# Autodesk Inventor assembly: for_bool
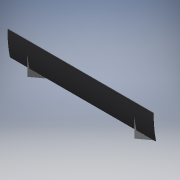
[picture p0: Inventor's stored thumbnail of the model, 180x180]
Saved by Autodesk Inventor 2018.1 (Build 221171000, 171)
## iProperties
Created: 2017-10-22
Part Number: for_bool
Material: 一般
Document SubType Name: Assembly
Designer: ku_sk
Author: ku_sk
## Documents named in this file (3)
- D:\kuwano\Documents\Inventor\KITformula\KS-15_Aero_CAD\type4\F-wing\parts\base\for_bool.iam
- D:\kuwano\Documents\Inventor\KITformula\KS-15_Aero_CAD\type4\F-wing\parts\base\base.ipt
- D:\kuwano\Documents\Inventor\KITformula\KS-15_Aero_CAD\type4\F-wing\parts\element_side\parts\stay_middle.ipt
## Components (3 placed, 2 different names)
1. base:1 — メイト:1, メイト:4, メイト:5, メイト:6, フラッシュ:3, フラッシュ:4, フラッシュ:5, フラッシュ:6
2. stay_middle:1 — メイト:1, メイト:5, フラッシュ:4
3. stay_middle:2 — メイト:4, メイト:6, フラッシュ:3
## Relationships (8: Mate 4, Flush 4)
- メイト:1 [Mate]: base:1 ↔ stay_middle:1
- メイト:4 [Mate]: base:1 ↔ stay_middle:2
- メイト:5 [Mate]: base:1 ↔ stay_middle:1
- メイト:6 [Mate]: base:1 ↔ stay_middle:2
- フラッシュ:3 [Flush] (180 mm): base:1 ↔ stay_middle:2
- フラッシュ:4 [Flush] (180 mm): base:1 ↔ stay_middle:1
- フラッシュ:5 [Flush]: base:1
- フラッシュ:6 [Flush]: base:1
